# Autodesk Inventor assembly: Tank Drive
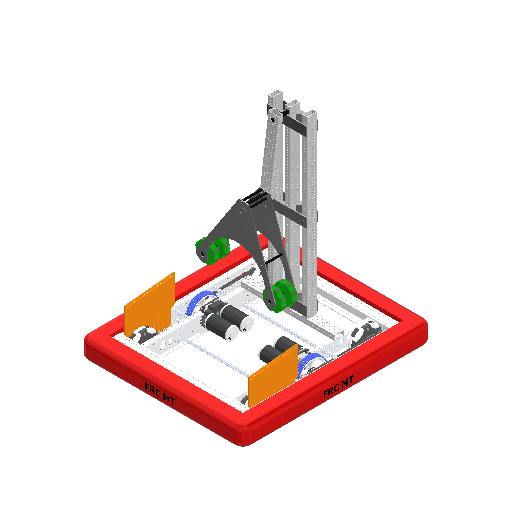
[picture p0: Inventor's stored thumbnail of the model, 512x512]
Saved by Autodesk Inventor 2027.1 (Build 311270010, 270A)
## iProperties
Created: 2026-08-13
Part Number: Tank Drive
Document SubType Name: Assembly
Designer: djair.oliveira
Author: djair.oliveira
## Documents named in this file (4)
- C:\Users\djair.oliveira\Documents\GitHub\MT_2026\CAD\Model C\Tank Drive.iam
- C:\Users\djair.oliveira\Documents\GitHub\MT_2026\CAD\Model C\AM14U5 Long ToughBox Mini 6in HiGrip 6wD v5\AM14U5 Long ToughBox Mini 6in HiGrip 6wD v5.iam
- C:\Users\djair.oliveira\Documents\GitHub\MT_2026\CAD\Model C\Elevador\Forja - Move Elevador.ipt
- C:\Users\djair.oliveira\Documents\GitHub\MT_2026\CAD\Model C\Hand\Hand.iam
## Components (3 placed, 3 different names)
1. AM14U5 Long ToughBox Mini 6in HiGrip 6wD v5:1 [sub-assembly] — Coincidente:1, Alinhado:3, Alinhado:4, Coincidente:2, Coincidente:3, Coincidente:4
2. Forja - Move Elevador:1 — Coincidente:2, Coincidente:3, Coincidente:4, Coincidente:5, Coincidente:6
3. Hand:1 [sub-assembly] — Coincidente:5, Coincidente:6
## Relationships (8: Mate 6, Flush 2)
- Coincidente:1 [Mate] (50 mm): AM14U5 Long ToughBox Mini 6in HiGrip 6wD v5:1
- Alinhado:3 [Flush] (412.337 mm): AM14U5 Long ToughBox Mini 6in HiGrip 6wD v5:1
- Alinhado:4 [Flush] (344.9 mm): AM14U5 Long ToughBox Mini 6in HiGrip 6wD v5:1
- Coincidente:2 [Mate]: AM14U5 Long ToughBox Mini 6in HiGrip 6wD v5:1 ↔ Forja - Move Elevador:1
- Coincidente:3 [Mate]: AM14U5 Long ToughBox Mini 6in HiGrip 6wD v5:1 ↔ Forja - Move Elevador:1
- Coincidente:4 [Mate]: AM14U5 Long ToughBox Mini 6in HiGrip 6wD v5:1 ↔ Forja - Move Elevador:1
- Coincidente:5 [Mate]: Forja - Move Elevador:1 ↔ Hand:1
- Coincidente:6 [Mate]: Forja - Move Elevador:1 ↔ Hand:1
